# Autodesk Inventor assembly: bachi_v4
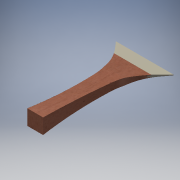
[picture p0: Inventor's stored thumbnail of the model, 180x180]
Saved by Autodesk Inventor 2019 (Build 230136000, 136)
## iProperties
Created: 2021-02-08
Part Number: bachi_v4
Material: Типовые
Document SubType Name: Assembly
Designer: stepa
Mass: 45.3977 g
Surface Area: 192.055 cm^2
Volume: 64.4113 cm^3
Density: 0.70481 g/cm^3
Author: stepa
## Documents named in this file (3)
- C:\Users\stepa\Documents\Inventor\Shamisen\bachi_v4.iam
- C:\Users\stepa\Documents\Inventor\Shamisen\bachi_v4.ipt
- C:\Users\stepa\Documents\Inventor\Shamisen\bachi_v4_1.ipt
## Components (2 placed, 2 different names)
1. bachi_v4:1 — Совмещение:1, Совмещение:2, Совмещение:3
2. bachi_v4_1:1 — Совмещение:1, Совмещение:2, Совмещение:3
## Relationships (3: Mate 3)
- Совмещение:1 [Mate]: bachi_v4:1 ↔ bachi_v4_1:1
- Совмещение:2 [Mate]: bachi_v4:1 ↔ bachi_v4_1:1
- Совмещение:3 [Mate]: bachi_v4:1 ↔ bachi_v4_1:1
